# Autodesk Inventor assembly: fullAssy
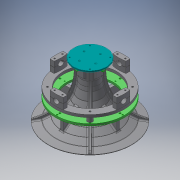
[picture p0: Inventor's stored thumbnail of the model, 180x180]
Saved by Autodesk Inventor 2016 SP1 (Build 200210100, 210)
## iProperties
Created: 2016-01-13
Part Number: fullAssy
Document SubType Name: Assembly
Designer: ddeboer
Author: ddeboer
## Documents named in this file (3)
- C:\Users\ddeboer\Desktop\leuschner-cad\fullAssy.iam
- C:\Users\ddeboer\Desktop\leuschner-cad\fixedMount.iam
- C:\Users\ddeboer\Desktop\leuschner-cad\feed.iam
## Components (2 placed, 2 different names)
1. fixedMount:1 [sub-assembly] — Insert:1
2. feed:1 [sub-assembly] — Insert:1
## Relationships (1: Insert 1)
- Insert:1 (25.4 mm): fixedMount:1 ↔ feed:1
